# Autodesk Inventor assembly: Z Axis FL
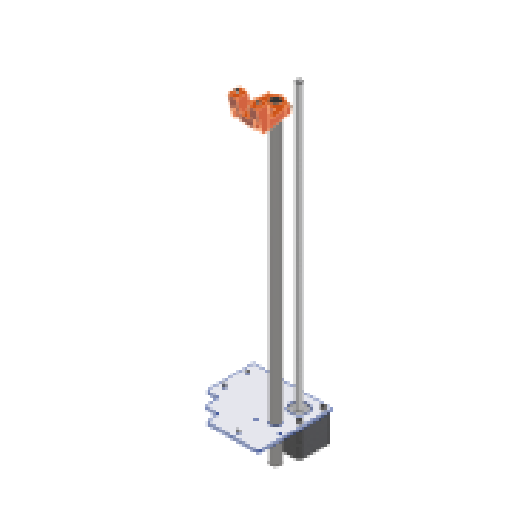
[picture p0: Inventor's stored thumbnail of the model, 512x512]
Saved by Autodesk Inventor 2023.2 (Build 272271000, 271)
## iProperties
Created: 2023-02-02
Part Number: Z Axis FL
Document SubType Name: Assembly
Designer: remop
Author: remop
## Documents named in this file (9)
- C:\Users\remop\OneDrive\Documents\Inventor\3D Printers\LuEVO\Mk5_FullKinematic\Z Axis Front Left.iam
- C:\Users\remop\OneDrive\Documents\Inventor\3D Printers\LuEVO\Mk5_FullKinematic\Z Axis Side Motor Mount.ipt
- C:\Users\remop\OneDrive\Documents\Inventor\3D Printers\LuEVO\Mk5_FullKinematic\Z Axis Guide.ipt
- C:\Users\remop\OneDrive\Documents\Inventor\3D Printers\LuEVO\Mk5_FullKinematic\Z Axis Motor.ipt
- C:\Users\remop\OneDrive\Documents\Inventor\3D Printers\LuEVO\Mk5_FullKinematic\Z Axis Top Brace.ipt
- C:\Users\remop\OneDrive\Documents\Inventor\Content Center Files\R2023\en-US\AS 1420\AS 1420 - 1973 - M3 x 6.ipt
- C:\Users\remop\OneDrive\Documents\Inventor\Content Center Files\R2023\en-US\AS 1420\AS 1420 - 1973 - M3 x 8.ipt
- C:\Users\remop\OneDrive\Documents\Inventor\3D Printers\LuEVO\Mk5_FullKinematic\Z Axis Top Brace Clamp.ipt
- C:\Users\remop\OneDrive\Documents\Inventor\Content Center Files\R2023\en-US\AS 1420\AS 1420 - 1973 - M3 x 12.ipt
## Components (16 placed, 8 different names)
1. Z Axis Side Motor Mount:1 — Rigid:1, Rigid:2, Angle:1, Insert:1, Insert:2, Insert:3, Insert:4, Insert:5, Insert:6, Insert:7
2. Z Axis Guide:1 — Rigid:2, Mate:1, Flush:1
3. Z Axis Motor:1 — Rigid:1
4. Z Axis Top Brace:1 — Mate:1, Angle:1, Flush:1, Insert:8, Insert:9, Rigid:4
5. AS 1420 - Metric M3 x 6:1 — Insert:1
6. AS 1420 - Metric M3 x 6:2 — Insert:2
7. AS 1420 - Metric M3 x 6:3 — Insert:3
8. AS 1420 - Metric M3 x 6:4 — Insert:4
9. AS 1420 - Metric M3 x 6:5 — Insert:5
10. AS 1420 - Metric M3 x 6:6 — Insert:6
11. AS 1420 - Metric M3 x 6:7 — Insert:7
12. AS 1420 - Metric M3 x 8:1 — Insert:8
13. AS 1420 - Metric M3 x 8:2 — Insert:9
14. Z Axis Top Brace Clamp:1 — Rigid:4
15. AS 1420 - Metric M3 x 12:1
16. AS 1420 - Metric M3 x 12:2
## Relationships (17: Insert 10, WeldJoint 4, Mate 1, Angle 1, Flush 1)
- Rigid:1 [WeldJoint]: Z Axis Side Motor Mount:1 ↔ Z Axis Motor:1
- Rigid:2 [WeldJoint] (-45 mm): Z Axis Side Motor Mount:1 ↔ Z Axis Guide:1
- Mate:1: Z Axis Guide:1 ↔ Z Axis Top Brace:1
- Angle:1 (90 deg): Z Axis Side Motor Mount:1 ↔ Z Axis Top Brace:1
- Flush:1: Z Axis Guide:1 ↔ Z Axis Top Brace:1
- Insert:1: Z Axis Side Motor Mount:1 ↔ AS 1420 - Metric M3 x 6:1
- Insert:2: Z Axis Side Motor Mount:1 ↔ AS 1420 - Metric M3 x 6:2
- Insert:3: Z Axis Side Motor Mount:1 ↔ AS 1420 - Metric M3 x 6:3
- Insert:4: Z Axis Side Motor Mount:1 ↔ AS 1420 - Metric M3 x 6:4
- Insert:5: Z Axis Side Motor Mount:1 ↔ AS 1420 - Metric M3 x 6:5
- Insert:6: Z Axis Side Motor Mount:1 ↔ AS 1420 - Metric M3 x 6:6
- Insert:7: Z Axis Side Motor Mount:1 ↔ AS 1420 - Metric M3 x 6:7
- Insert:8: Z Axis Top Brace:1 ↔ AS 1420 - Metric M3 x 8:1
- Insert:9: Z Axis Top Brace:1 ↔ AS 1420 - Metric M3 x 8:2
- [Insert]: Z Axis Top Brace Clamp:1 ↔ AS 1420 - Metric M3 x 12:1
- [WeldJoint]: Z Axis Top Brace Clamp:1 ↔ AS 1420 - Metric M3 x 12:2
- Rigid:4 [WeldJoint]: Z Axis Top Brace:1 ↔ Z Axis Top Brace Clamp:1
## Named parameters: d38_d39 = 0 mm, d39_d40 = 0 mm, d40_d41 = 0 mm
